# Autodesk Inventor assembly: TAMIYA_6-SpeedGearBox
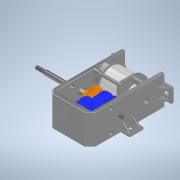
[picture p0: Inventor's stored thumbnail of the model, 180x180]
Saved by Autodesk Inventor 2022.3 (Build 263350000, 350)
## iProperties
Created: 2020-05-27
Part Number: TAMIYA_6-SpeedGearBox
Document SubType Name: Assembly
Designer: Hagihara Yuya
Mass: 112.287 g
Surface Area: 263.822 cm^2
Volume: 37.2906 cm^3
Density: 3.01112 g/cm^3
Author: Hagihara Yuya
## Documents named in this file (10)
- C:\Users\YusukeKunita\Documents\GrabCAD\Development\BasicParts\TAMIYA_6-SpeedGearBox\TAMIYA_6-SpeedGearBox.iam
- C:\Users\YusukeKunita\Documents\GrabCAD\Development\BasicParts\TAMIYA_6-SpeedGearBox\GearBox.ipt
- C:\Users\YusukeKunita\Documents\GrabCAD\Development\BasicParts\TAMIYA_6-SpeedGearBox\GearShaft_1.ipt
- C:\Users\YusukeKunita\Documents\GrabCAD\Development\BasicParts\TAMIYA_6-SpeedGearBox\GearShaft_2.ipt
- C:\Users\YusukeKunita\Documents\GrabCAD\Development\BasicParts\TAMIYA_6-SpeedGearBox\Motor_230.ipt
- C:\Users\YusukeKunita\Documents\GrabCAD\Development\BasicParts\TAMIYA_6-SpeedGearBox\TAMIYA_6-SpeedGearBox\デザイン アクセラレータ\平歯車1.iam
- C:\Users\YusukeKunita\Documents\GrabCAD\Development\BasicParts\TAMIYA_6-SpeedGearBox\TAMIYA_6-SpeedGearBox\デザイン アクセラレータ\平歯車2.iam
- C:\Users\YusukeKunita\Documents\GrabCAD\Development\BasicParts\TAMIYA_6-SpeedGearBox\GearShaft_3.ipt
- C:\Users\YusukeKunita\Documents\GrabCAD\Development\BasicParts\TAMIYA_6-SpeedGearBox\TAMIYA_6-SpeedGearBox\デザイン アクセラレータ\平歯車3.iam
- C:\Users\YusukeKunita\Documents\GrabCAD\Development\BasicParts\TAMIYA_6-SpeedGearBox\TAMIYA_6-SpeedGearBox\デザイン アクセラレータ\平歯車4.iam
## Components (17 placed, 6 different names)
1. GearBox:1 — 回転:1, 回転:5, フラッシュ:2, 円柱状:1, 回転:8, 回転:9, 回転:10
2. GearShaft_1:1 — フラッシュ:2, 円柱状:1
3. GearShaft_2:1 — 回転:8
4. GearShaft_3:1 — 回転:5, 回転:6
5. Motor_230:1 — 回転:1, メイト:6, フラッシュ:1
6. 平歯車:1 [sub-assembly] — リジッド:1, メイト:4, メイト:5, 回転:2, 回転:10
7. 平歯車:10 [sub-assembly]
8. 平歯車:11 [sub-assembly] — 回転:6, メイト:4, 回転:1
9. 平歯車:12 [sub-assembly] — 回転:2
10. 平歯車:13 [sub-assembly] — 回転:7
11. 平歯車:14 [sub-assembly] — メイト:6, フラッシュ:1, 回転:1
12. 平歯車:2 [sub-assembly] — リジッド:1, 回転:2, 回転:3
13. 平歯車:5 [sub-assembly] — 回転:2, 回転:4
14. 平歯車:6 [sub-assembly] — 回転:5, 回転:7
15. 平歯車:7 [sub-assembly] — メイト:5, 回転:3, 回転:9
16. 平歯車:8 [sub-assembly] — 回転:4, 回転:4
17. 平歯車:9 [sub-assembly] — 回転:4, 回転:5
## Relationships (25: RevoluteJoint 9, WeldJoint 5, RelateRotation 5, Mate 3, Flush 2, CylindricalJoint 1)
- 回転:1 [RevoluteJoint]: GearBox:1 ↔ Motor_230:1
- リジッド:1 [WeldJoint]: 平歯車:1 ↔ 平歯車:2
- [WeldJoint]: 平歯車:5 ↔ 平歯車:6
- [WeldJoint]: 平歯車:7 ↔ 平歯車:8
- [WeldJoint]: 平歯車:10 ↔ 平歯車:9
- [WeldJoint]: 平歯車:11 ↔ 平歯車:12
- 回転:2 [RevoluteJoint]: 平歯車:2 ↔ 平歯車:5
- 回転:4 [RevoluteJoint]: 平歯車:8 ↔ 平歯車:9
- 回転:5 [RevoluteJoint]: GearBox:1 ↔ GearShaft_3:1
- 回転:6 [RevoluteJoint]: GearShaft_3:1 ↔ 平歯車:11
- メイト:4 [Mate] (1 mm): 平歯車:1 ↔ 平歯車:11
- メイト:5 [Mate] (1 mm): 平歯車:1 ↔ 平歯車:7
- メイト:6 [Mate]: Motor_230:1 ↔ 平歯車:14
- フラッシュ:1 [Flush]: Motor_230:1 ↔ 平歯車:14
- 回転:1 [RelateRotation] (0.2222 ul): 平歯車:11 ↔ 平歯車:14
- 回転:2 [RelateRotation] (0.3889 ul): 平歯車:1 ↔ 平歯車:12
- 回転:3 [RelateRotation] (0.3889 ul): 平歯車:2 ↔ 平歯車:7
- 回転:4 [RelateRotation] (0.3889 ul): 平歯車:5 ↔ 平歯車:8
- 回転:5 [RelateRotation] (0.3889 ul): 平歯車:6 ↔ 平歯車:9
- フラッシュ:2 [Flush] (29 mm): GearBox:1 ↔ GearShaft_1:1
- 回転:7 [RevoluteJoint]: 平歯車:13 ↔ 平歯車:6
- 円柱状:1 [CylindricalJoint]: GearBox:1 ↔ GearShaft_1:1
- 回転:8 [RevoluteJoint]: GearBox:1 ↔ GearShaft_2:1
- 回転:9 [RevoluteJoint]: GearBox:1 ↔ 平歯車:7
- 回転:10 [RevoluteJoint]: GearBox:1 ↔ 平歯車:1
## Named parameters: d12_d10 = 0 mm, d13_d10 = 0 mm, d14_d10 = 0 mm, d15_d10 = 0 mm
